# Autodesk Inventor assembly: Nozzle_Assembly
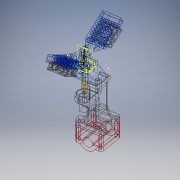
[picture p0: Inventor's stored thumbnail of the model, 180x180]
Saved by Autodesk Inventor 2016 (Build 200138000, 138)
## iProperties
Created: 2017-02-05
Part Number: Nozzle_Assembly
Document SubType Name: Assembly
Designer: Liquid Metal Printer
Author: Liquid Metal Printer
## Documents named in this file (14)
- C:\Users\Liquid Metal Printer\Desktop\Silicone Printer\CAD files\Extruder\Extruder\Nozzle\Extruder_Assembly.iam
- C:\Users\Liquid Metal Printer\Desktop\Silicone Printer\CAD files\Extruder\Extruder\Nozzle\Middle.ipt
- C:\Users\Liquid Metal Printer\Desktop\Silicone Printer\CAD files\Extruder\Extruder\Nozzle\Roof.ipt
- C:\Users\Liquid Metal Printer\Desktop\Silicone Printer\CAD files\Extruder\Extruder\Nozzle\Pillar.ipt
- C:\Users\Liquid Metal Printer\Desktop\Silicone Printer\CAD files\Extruder\Extruder\Nozzle\Motor.ipt
- C:\Users\Liquid Metal Printer\Desktop\Silicone Printer\CAD files\Extruder\Extruder\Nozzle\Upper_Nozzle.ipt
- C:\Users\Liquid Metal Printer\Desktop\Silicone Printer\CAD files\Extruder\Extruder\Nozzle\Upper_Seal.ipt
- C:\Users\Liquid Metal Printer\Desktop\Silicone Printer\CAD files\Extruder\Extruder\Nozzle\Mixer.ipt
- C:\Users\Liquid Metal Printer\Desktop\Silicone Printer\CAD files\Extruder\Extruder\Nozzle\Coupler.ipt
- C:\Users\Liquid Metal Printer\Desktop\Silicone Printer\CAD files\Extruder\Extruder\Nozzle\Nozzle_With_Heater.ipt
- C:\Users\Liquid Metal Printer\Desktop\Silicone Printer\CAD files\Extruder\Extruder\Nozzle\Left_Wing.ipt
- C:\Users\Liquid Metal Printer\Desktop\Silicone Printer\CAD files\Extruder\Extruder\Nozzle\Right_Wing.ipt
- C:\Users\Liquid Metal Printer\Desktop\Silicone Printer\CAD files\Extruder\Extruder\Nozzle\Ceramic_Heater.ipt
- C:\Users\Liquid Metal Printer\Desktop\Silicone Printer\CAD files\Extruder\Extruder\Nozzle\Fan_30mm.ipt
## Components (15 placed, 13 different names)
1. Middle:1 — Mate:1, Flush:1, Flush:2, Mate:2, Mate:3, Mate:4, Mate:5, Mate:6, Mate:7, Mate:8, Mate:9, Mate:10
2. Roof:1 — Mate:1, Flush:1, Flush:2, Mate:2, Mate:3, Mate:4, Mate:5
3. Pillar:1 — Mate:6, Mate:7, Mate:8, Mate:9, Mate:10, Insert:1, Mate:11, Mate:12, Mate:13, Mate:22
4. Motor:1 — Insert:1, Mate:14, Mate:20
5. Upper_Nozzle:1 — Mate:11, Mate:12, Mate:13, Mate:14, Mate:15, Mate:16, Mate:17, Mate:18, Mate:19, Mate:23, Mate:24, Mate:25, Mate:26
6. Upper_Seal:1 — Mate:15, Mate:16, Mate:17
7. Mixer:1 — Mate:18, Mate:19, Mate:21
8. Coupler:1 — Mate:20, Mate:21, Mate:22
9. Nozzle_With_Heater:1 — Mate:23, Mate:24, Mate:25, Mate:26, Mate:29, Mate:30, Angle:1, Mate:31, Mate:32, Angle:2
10. Left_Wing:1 — Mate:27, Flush:3, Mate:31, Mate:32, Angle:2, Mate:33, Flush:6, Flush:7
11. Right_Wing:1 — Mate:28, Flush:4, Mate:29, Mate:30, Angle:1, Mate:34, Flush:5, Flush:8
12. Ceramic_Heater:1 — Mate:27, Flush:3
13. Fan_30mm:1 — Mate:34, Flush:5, Flush:8
14. Ceramic_Heater:2 — Mate:28, Flush:4
15. Fan_30mm:2 — Mate:33, Flush:6, Flush:7
## Relationships (45: Mate 34, Flush 8, Angle 2, Insert 1)
- Mate:1 (2 mm): Middle:1 ↔ Roof:1
- Flush:1: Middle:1 ↔ Roof:1
- Flush:2: Middle:1 ↔ Roof:1
- Mate:2: Middle:1 ↔ Roof:1
- Mate:3: Middle:1 ↔ Roof:1
- Mate:4: Middle:1 ↔ Roof:1
- Mate:5: Middle:1 ↔ Roof:1
- Mate:6 (3 mm): Middle:1 ↔ Pillar:1
- Mate:7: Middle:1 ↔ Pillar:1
- Mate:8: Middle:1 ↔ Pillar:1
- Mate:9: Middle:1 ↔ Pillar:1
- Mate:10: Middle:1 ↔ Pillar:1
- Insert:1: Pillar:1 ↔ Motor:1
- Mate:11: Pillar:1 ↔ Upper_Nozzle:1
- Mate:12: Pillar:1 ↔ Upper_Nozzle:1
- Mate:13: Pillar:1 ↔ Upper_Nozzle:1
- Mate:14: Motor:1 ↔ Upper_Nozzle:1
- Mate:15: Upper_Nozzle:1 ↔ Upper_Seal:1
- Mate:16: Upper_Nozzle:1 ↔ Upper_Seal:1
- Mate:17: Upper_Nozzle:1 ↔ Upper_Seal:1
- Mate:18: Upper_Nozzle:1 ↔ Mixer:1
- Mate:19: Upper_Nozzle:1 ↔ Mixer:1
- Mate:20: Motor:1 ↔ Coupler:1
- Mate:21: Mixer:1 ↔ Coupler:1
- Mate:22 (3 mm): Pillar:1 ↔ Coupler:1
- Mate:23: Upper_Nozzle:1 ↔ Nozzle_With_Heater:1
- Mate:24: Upper_Nozzle:1 ↔ Nozzle_With_Heater:1
- Mate:25: Upper_Nozzle:1 ↔ Nozzle_With_Heater:1
- Mate:26: Upper_Nozzle:1 ↔ Nozzle_With_Heater:1
- Mate:27: Left_Wing:1 ↔ Ceramic_Heater:1
- Mate:28: Right_Wing:1 ↔ Ceramic_Heater:2
- Flush:3: Left_Wing:1 ↔ Ceramic_Heater:1
- Flush:4: Right_Wing:1 ↔ Ceramic_Heater:2
- Mate:29: Nozzle_With_Heater:1 ↔ Right_Wing:1
- Mate:30: Nozzle_With_Heater:1 ↔ Right_Wing:1
- Angle:1 (30 deg): Nozzle_With_Heater:1 ↔ Right_Wing:1
- Mate:31: Nozzle_With_Heater:1 ↔ Left_Wing:1
- Mate:32: Nozzle_With_Heater:1 ↔ Left_Wing:1
- Angle:2 (30 deg): Nozzle_With_Heater:1 ↔ Left_Wing:1
- Mate:33: Left_Wing:1 ↔ Fan_30mm:2
- Mate:34: Right_Wing:1 ↔ Fan_30mm:1
- Flush:5: Right_Wing:1 ↔ Fan_30mm:1
- Flush:6: Left_Wing:1 ↔ Fan_30mm:2
- Flush:7 (8 mm): Left_Wing:1 ↔ Fan_30mm:2
- Flush:8 (-8 mm): Right_Wing:1 ↔ Fan_30mm:1
